# Autodesk Inventor assembly: battery_status_monitor
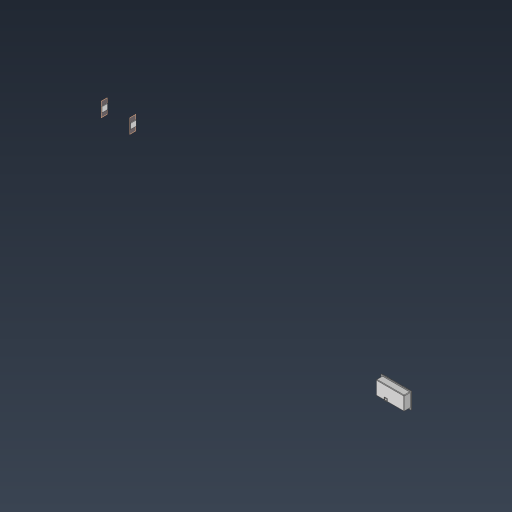
[picture p0: Inventor's stored thumbnail of the model, 512x512]
Saved by Autodesk Inventor 2023 (Build 270158000, 158)
## iProperties
Created: 2025-12-26
Part Number: battery_status_monitor
Document SubType Name: Assembly
Designer: szymo
Author: szymo
## Documents named in this file (4)
- D:\tech\diy\e-skateboard\projekcik-inventor\battery_status_monitor.iam
- **D:\tech\diy\e-skateboard\projekcik-inventor\main.iam*LocalDocs*xAaaaqgbaAaaaaaaaAaaaa0zdHc*DIY.ipt
- D:\tech\diy\e-skateboard\projekcik-inventor\piny_led_bateryjki.ipt
- D:\tech\diy\e-skateboard\projekcik-inventor\DIY.ipt
## Components (4 placed, 2 different names)
1. DIY:1 — Flush:1, Flush:2, Mate:1, Mate:2, Flush:3
2. piny_led_bateryjki:1 — Flush:1, Flush:2
3. piny_led_bateryjki:2 — Mate:1, Mate:2, Flush:3
4. DIY:2
## Relationships (5: Flush 3, Mate 2)
- Flush:1: DIY:1 ↔ piny_led_bateryjki:1
- Flush:2: DIY:1 ↔ piny_led_bateryjki:1
- Mate:1: DIY:1 ↔ piny_led_bateryjki:2
- Mate:2: DIY:1 ↔ piny_led_bateryjki:2
- Flush:3 (8.75 mm): DIY:1 ↔ piny_led_bateryjki:2
